# Autodesk Inventor assembly: CE-5.1.1
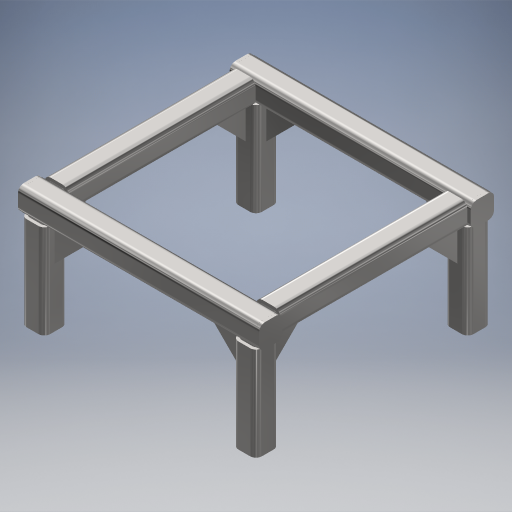
[picture p0: Inventor's stored thumbnail of the model, 512x512]
Saved by Autodesk Inventor 2024 (Build 280153000, 153)
## iProperties
_SolveAssemblyDoc: Frame Generator Solve Assembly
_Version: 25.0.0
Created: 2024-02-08
Part Number: CE-5.1.1
Document SubType Name: Assembly
Designer: Alex
Author: Alex
## Documents named in this file (4)
- C:\Shared\alex-bartella-schoolwork\4z03\Week 4\CE-5.1.1.iam
- C:\Shared\alex-bartella-schoolwork\4z03\Week 4\CE-5.1.1\CE-5.1.1-00.ipt
- C:\Shared\alex-bartella-schoolwork\4z03\Week 4\CE-5.1.1\CE-5.1.1-00.iam
- C:\Shared\alex-bartella-schoolwork\4z03\Week 4\CE-5.1.1\CE-5.1.1-10.ipt
## Components (10 placed, 2 different names)
1. CE-5.1.1-00:1
2. CE-5.1.1-00:2 [sub-assembly] — Mate:1, Mate:2, Mate:3, Mate:4, Mate:5, Mate:6, Mate:7, Mate:8, Mate:9, Mate:10, Mate:11, Mate:12, Mate:13, Mate:14, Mate:15, Mate:16, Mate:17, Angle:1, Mate:18, Angle:2, Mate:19, Angle:3, Mate:20, Angle:4
3. CE-5.1.1-10:1 — Mate:1, Mate:2, Mate:21
4. CE-5.1.1-10:2 — Mate:3, Mate:4, Mate:22
5. CE-5.1.1-10:3 — Mate:5, Mate:6, Flush:1
6. CE-5.1.1-10:4 — Mate:7, Mate:8, Flush:2
7. CE-5.1.1-10:5 — Mate:9, Mate:10, Mate:23
8. CE-5.1.1-10:6 — Mate:11, Mate:12, Flush:3
9. CE-5.1.1-10:7 — Mate:13, Mate:14, Mate:24
10. CE-5.1.1-10:8 — Mate:15, Mate:16, Flush:4
## Relationships (32: Mate 24, Angle 4, Flush 4)
- Mate:1: CE-5.1.1-00:2 ↔ CE-5.1.1-10:1
- Mate:2: CE-5.1.1-00:2 ↔ CE-5.1.1-10:1
- Mate:3: CE-5.1.1-00:2 ↔ CE-5.1.1-10:2
- Mate:4: CE-5.1.1-00:2 ↔ CE-5.1.1-10:2
- Mate:5: CE-5.1.1-00:2 ↔ CE-5.1.1-10:3
- Mate:6: CE-5.1.1-00:2 ↔ CE-5.1.1-10:3
- Mate:7: CE-5.1.1-00:2 ↔ CE-5.1.1-10:4
- Mate:8: CE-5.1.1-00:2 ↔ CE-5.1.1-10:4
- Mate:9: CE-5.1.1-00:2 ↔ CE-5.1.1-10:5
- Mate:10: CE-5.1.1-00:2 ↔ CE-5.1.1-10:5
- Mate:11: CE-5.1.1-00:2 ↔ CE-5.1.1-10:6
- Mate:12: CE-5.1.1-00:2 ↔ CE-5.1.1-10:6
- Mate:13: CE-5.1.1-00:2 ↔ CE-5.1.1-10:7
- Mate:14: CE-5.1.1-00:2 ↔ CE-5.1.1-10:7
- Mate:15: CE-5.1.1-00:2 ↔ CE-5.1.1-10:8
- Mate:16: CE-5.1.1-00:2 ↔ CE-5.1.1-10:8
- Mate:17: CE-5.1.1-00:2
- Angle:1 (0 deg): CE-5.1.1-00:2
- Mate:18: CE-5.1.1-00:2
- Angle:2 (0 deg): CE-5.1.1-00:2
- Mate:19: CE-5.1.1-00:2
- Angle:3 (0 deg): CE-5.1.1-00:2
- Mate:20: CE-5.1.1-00:2
- Angle:4 (0 deg): CE-5.1.1-00:2
- Mate:21: CE-5.1.1-10:1
- Mate:22: CE-5.1.1-10:2
- Flush:1: CE-5.1.1-10:3
- Flush:2: CE-5.1.1-10:4
- Mate:23: CE-5.1.1-10:5
- Flush:3: CE-5.1.1-10:6
- Mate:24: CE-5.1.1-10:7
- Flush:4: CE-5.1.1-10:8
